# Autodesk Inventor assembly: washerAndThrustBearingAssembly
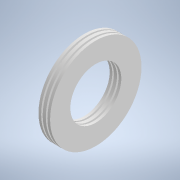
[picture p0: Inventor's stored thumbnail of the model, 180x180]
Saved by Autodesk Inventor 2020.2 (Build 242310000, 310)
## iProperties
Created: 2020-01-07
Part Number: washerAndThrustBearingAssembly
Document SubType Name: Assembly
Designer: steele
Author: steele
## Documents named in this file (3)
- C:\git\CAD-Development\robSteele\2020 Lift Mechanism\washerAndThrustBearingAssembly.iam
- C:\git\CAD-Development\robSteele\2020 Lift Mechanism\5909K320_THRUST NEEDLE-ROLLER BEARING.ipt
- C:\git\CAD-Development\robSteele\2020 Lift Mechanism\5909K450_THRUST NEEDLE-ROLLER BEARING.ipt
## Components (3 placed, 2 different names)
1. 5909K320_THRUST NEEDLE-ROLLER BEARING:1 — Insert:1, Insert:2
2. 5909K450_THRUST NEEDLE-ROLLER BEARING:1 — Insert:1
3. 5909K450_THRUST NEEDLE-ROLLER BEARING:2 — Insert:2
## Relationships (2: Insert 2)
- Insert:1 (0.508 mm): 5909K320_THRUST NEEDLE-ROLLER BEARING:1 ↔ 5909K450_THRUST NEEDLE-ROLLER BEARING:1
- Insert:2 (0.508 mm): 5909K320_THRUST NEEDLE-ROLLER BEARING:1 ↔ 5909K450_THRUST NEEDLE-ROLLER BEARING:2
